# Autodesk Inventor assembly: 0.5in_tnut
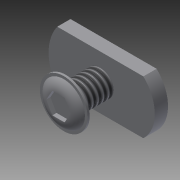
[picture p0: Inventor's stored thumbnail of the model, 180x180]
Saved by Autodesk Inventor 2014 (Build 180170000, 170)
## iProperties
Created: 2014-10-05
Part Number: 0.5in_tnut
Document SubType Name: Assembly
Designer: Matthew
Author: Matthew
## Documents named in this file (3)
- C:\Users\Matthew\Documents\GitHub\CNC Mill\8020\0.5in_tnut.iam
- C:\Users\Matthew\Documents\GitHub\CNC Mill\8020\3786_economy_slide_tnuts.ipt
- C:\Users\Matthew\Documents\GitHub\CNC Mill\8020\8020_10series_0.5in_0.25-20_capscrews.ipt
## Components (2 placed, 2 different names)
1. 3786_economy_slide_tnuts:1 — Insert:1
2. 8020_10series_0.5in_0.25-20_capscrews:1 — Insert:1
## Relationships (1: Insert 1)
- Insert:1: 3786_economy_slide_tnuts:1 ↔ 8020_10series_0.5in_0.25-20_capscrews:1
